# Autodesk Inventor assembly: Aktor_neu
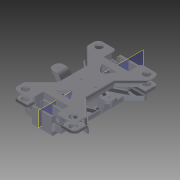
[picture p0: Inventor's stored thumbnail of the model, 180x180]
Saved by Autodesk Inventor 2015 (Build 190159000, 159)
## iProperties
Created: 2017-10-10
Part Number: Aktor_neu
Document SubType Name: Assembly
Designer: Wilczynski
Author: Wilczynski
## Documents named in this file (3)
- M:\Aktoren\Version3\Aktor_neu.iam
- M:\Aktoren\Version3\Platte.ipt
- M:\Aktoren\Version3\PlatteOben.ipt
## Components (2 placed, 2 different names)
1. Platte:1 — Passend:1, Passend:2
2. PlatteOben:1 — Passend:1, Passend:2
## Relationships (2: Mate 2)
- Passend:1 [Mate] (13 mm): Platte:1 ↔ PlatteOben:1
- Passend:2 [Mate]: Platte:1 ↔ PlatteOben:1
